# Autodesk Inventor assembly: XM430_ASM_WITHOUT-BACK
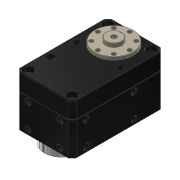
[picture p0: Inventor's stored thumbnail of the model, 180x180]
Saved by Autodesk Inventor 2019.4 (Build 234330000, 330)
## iProperties
Created: 2019-10-08
Part Number: XM430_ASM_WITHOUT-BACK
Material: 一般
Document SubType Name: Assembly
Designer: y6tada
Author: y6tada
## Documents named in this file (4)
- C:\Workspace\Yuni8\Libs\DYNAMIXEL\XM430\XM430_ASM_WITHOUT-BACK.iam
- C:\Workspace\Yuni8\Libs\DYNAMIXEL\XM430\XM430_HOUSING_MIDDLE.ipt
- C:\Workspace\Yuni8\Libs\DYNAMIXEL\XM430\XM430_HOUSING_TOP.ipt
- C:\Workspace\Yuni8\Libs\DYNAMIXEL\XM430\XM430_HORN.ipt
## Components (3 placed, 3 different names)
1. XM430_HOUSING_MIDDLE:1 — フラッシュ:1, フラッシュ:2, フラッシュ:3, フラッシュ:4, フラッシュ:5, メイト:1
2. XM430_HOUSING_TOP:1 — フラッシュ:4, フラッシュ:5, メイト:1, メイト:2, メイト:3, フラッシュ:6
3. XM430_HORN:1 — メイト:2, メイト:3, フラッシュ:6
## Relationships (9: Flush 6, Mate 3)
- フラッシュ:1 [Flush]: XM430_HOUSING_MIDDLE:1
- フラッシュ:2 [Flush]: XM430_HOUSING_MIDDLE:1
- フラッシュ:3 [Flush]: XM430_HOUSING_MIDDLE:1
- フラッシュ:4 [Flush]: XM430_HOUSING_MIDDLE:1 ↔ XM430_HOUSING_TOP:1
- フラッシュ:5 [Flush]: XM430_HOUSING_MIDDLE:1 ↔ XM430_HOUSING_TOP:1
- メイト:1 [Mate]: XM430_HOUSING_MIDDLE:1 ↔ XM430_HOUSING_TOP:1
- メイト:2 [Mate]: XM430_HOUSING_TOP:1 ↔ XM430_HORN:1
- メイト:3 [Mate]: XM430_HOUSING_TOP:1 ↔ XM430_HORN:1
- フラッシュ:6 [Flush]: XM430_HOUSING_TOP:1 ↔ XM430_HORN:1
